# Autodesk Inventor assembly: メカオンリーiam
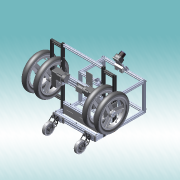
[picture p0: Inventor's stored thumbnail of the model, 180x180]
Saved by Autodesk Inventor 2015 (Build 190159000, 159)
## iProperties
Created: 2016-02-29
Part Number: メカオンリーiam
Document SubType Name: Assembly
Designer: buzztaka
Author: buzztaka
## Documents named in this file (51)
- C:\Users\buzztaka\Documents\tukuba\i-cart-middle_3d-model\計測輪アセンブル\メカオンリーiam.iam
- C:\Users\buzztaka\Documents\tukuba\i-cart-middle_3d-model\計測輪アセンブル\wheel_12inch.ipt
- C:\Users\buzztaka\Documents\tukuba\i-cart-middle_3d-model\計測輪アセンブル\wheel-cap.ipt
- C:\Users\buzztaka\Documents\tukuba\i-cart-middle_3d-model\計測輪アセンブル\wheel-hub.ipt
- C:\Users\buzztaka\Documents\tukuba\i-cart-middle_3d-model\計測輪アセンブル\HFS60A5-20-70.ipt
- C:\Users\buzztaka\Documents\tukuba\i-cart-middle_3d-model\計測輪アセンブル\HBLBL5.ipt
- C:\Users\buzztaka\Documents\tukuba\i-cart-middle_3d-model\計測輪アセンブル\hblfsn5.ipt
- C:\Users\buzztaka\Documents\tukuba\i-cart-middle_3d-model\計測輪アセンブル\hblfsnf5.ipt
- C:\Users\buzztaka\Documents\tukuba\i-cart-middle_3d-model\計測輪アセンブル\HBLFSSW5.ipt
- C:\Users\buzztaka\Documents\tukuba\i-cart-middle_3d-model\計測輪アセンブル\hntaj5_5.ipt
- C:\Users\buzztaka\Documents\tukuba\i-cart-middle_3d-model\計測輪アセンブル\UST-20LX.ipt
- C:\Users\buzztaka\Documents\tukuba\i-cart-middle_3d-model\計測輪アセンブル\MTi-30.ipt
- C:\Users\buzztaka\Documents\tukuba\i-cart-middle_3d-model\計測輪アセンブル\HFSB5-2020-550-LCH-RWV-AH30-BH240-CH280-DH442-EH462.ipt
- C:\Users\buzztaka\Documents\tukuba\i-cart-middle_3d-model\計測輪アセンブル\CAF5-2020-432-LCH-RCH-AH167-BH217.ipt
- C:\Users\buzztaka\Documents\tukuba\i-cart-middle_3d-model\計測輪アセンブル\エンコーダ取り付け.iam
- C:\Users\buzztaka\Documents\tukuba\i-cart-middle_3d-model\計測輪アセンブル\HFSB5-2020-80-TPW.ipt
- C:\Users\buzztaka\Documents\tukuba\i-cart-middle_3d-model\計測輪アセンブル\CAF5-2040-432-LCH-RCH-AH167-BH217切り出し後.ipt
- C:\Users\buzztaka\Documents\tukuba\i-cart-middle_3d-model\計測輪アセンブル\ힼ�ힼ�ힼ�ힼ�.ipt
- C:\Users\buzztaka\Documents\tukuba\i-cart-middle_3d-model\計測輪アセンブル\ힼ�ힼ�ힼ�ힼ�ힼ�-L1.ipt
- C:\Users\buzztaka\Documents\tukuba\i-cart-middle_3d-model\計測輪アセンブル\ힼ�ힼ�ힼ�ힼ�ힼ�-L2.ipt
- C:\Users\buzztaka\Documents\tukuba\i-cart-middle_3d-model\計測輪アセンブル\ힼ�ힼ�ힼ�ힼ�ힼ�-ힽ�ힽ�.ipt
- C:\Users\buzztaka\Documents\tukuba\i-cart-middle_3d-model\計測輪アセンブル\ힼ�ힼ�ힼ�ힼ�ힼ�-ힼ�ힽ�ힽ�.ipt
- C:\Users\buzztaka\Documents\tukuba\i-cart-middle_3d-model\計測輪アセンブル\ힼ�ힼ�ힼ�ힼ�-ힼ�ힽ�ힽ�Lힼ�ힼ�ힼ�ힼ�ힼ�.ipt
- C:\Users\buzztaka\Documents\tukuba\i-cart-middle_3d-model\計測輪アセンブル\ힼ�ힼ�ힼ�ힼ�ힼ�-ힼ�ힼ�ힼ�ힼ�ힼ�ힽ�ힼ�ힼ�ힽ�.ipt
- C:\Users\buzztaka\Documents\tukuba\i-cart-middle_3d-model\計測輪アセンブル\ힼ�ힼ�ힼ�ힼ�(ힽ�ힽ�).ipt
- C:\Users\buzztaka\Documents\tukuba\i-cart-middle_3d-model\計測輪アセンブル\ힼ�ힼ�ힼ�ힼ�ힼ�ힼ�ힼ�-2020-L2.ipt
- C:\Users\buzztaka\Documents\tukuba\i-cart-middle_3d-model\計測輪アセンブル\ힼ�ힼ�ힼ�ힼ�ힼ�ힼ�ힼ�-2040-L2.ipt
- C:\Users\buzztaka\Documents\tukuba\i-cart-middle_3d-model\計測輪アセンブル\ힼ�ힼ�ힼ�ힼ�ힼ�ힼ�ힼ�-2060-L2.ipt
- C:\Users\buzztaka\Documents\tukuba\i-cart-middle_3d-model\計測輪アセンブル\ힼ�ힼ�ힼ�ힼ�ힼ�ힼ�ힼ�-2040-L3.ipt
- C:\Users\buzztaka\Documents\tukuba\i-cart-middle_3d-model\計測輪アセンブル\ힼ�ힼ�ힼ�ힼ�ힼ�ힼ�ힼ�-2020-L4.ipt
- C:\Users\buzztaka\Documents\tukuba\i-cart-middle_3d-model\計測輪アセンブル\ힼ�ힼ�ힼ�ힼ�ힼ�ힼ�ힼ�-2020-L5.ipt
- C:\Users\buzztaka\Documents\tukuba\i-cart-middle_3d-model\計測輪アセンブル\ힼ�ힼ�ힼ�ힼ�ힼ�ힼ�ힼ�-2020-L6.ipt
- C:\Users\buzztaka\Documents\tukuba\i-cart-middle_3d-model\計測輪アセンブル\ힼ�ힼ�ힼ�ힼ�ힼ�ힼ�ힼ�-2020-L7.ipt
- C:\Users\buzztaka\Documents\tukuba\i-cart-middle_3d-model\計測輪アセンブル\ힼ�ힼ�ힼ�ힼ�ힼ�ힼ�ힼ�-ힽ�ힽ�ힽ�ힼ�ힼ�ힼ�ힼ�ힼ�ힼ�.ipt
- C:\Users\buzztaka\Documents\tukuba\i-cart-middle_3d-model\計測輪アセンブル\ힼ�ힼ�ힼ�ힼ�ힼ�ힼ�ힼ�-ힼ�ힼ�ힼ�-M5.ipt
- C:\Users\buzztaka\Documents\tukuba\i-cart-middle_3d-model\計測輪アセンブル\ힼ�ힼ�ힼ�ힼ�ힼ�ힼ�ힼ�-ힽ�ힼ�ힽ�ힼ�ힼ�.ipt
- C:\Users\buzztaka\Documents\tukuba\i-cart-middle_3d-model\計測輪アセンブル\URG_ힼ�ힽ�ힽ�ힼ�ힼ�ힼ�ힽ�.ipt
- C:\Users\buzztaka\Documents\tukuba\i-cart-middle_3d-model\計測輪アセンブル\imu_ힼ�ힼ�ힼ�ힼ�.ipt
- C:\Users\buzztaka\Documents\tukuba\i-cart-middle_3d-model\計測輪アセンブル\ힽ�ힼ�ힼ�ힼ�ힼ�ힽ�.ipt
- C:\Users\buzztaka\Documents\tukuba\i-cart-middle_3d-model\計測輪アセンブル\M3ힽ�ힼ�ힼ�ힼ�ힼ�ힼ�ힼ�.ipt
- C:\Users\buzztaka\Documents\tukuba\i-cart-middle_3d-model\計測輪アセンブル\ힼ�ힼ�ힼ�-M5.ipt
- C:\Users\buzztaka\Documents\tukuba\i-cart-middle_3d-model\計測輪アセンブル\ힼ�ힼ�-Cap-M5-12.ipt
- C:\Users\buzztaka\Documents\tukuba\i-cart-middle_3d-model\計測輪アセンブル\ힼ�ힼ�-Cap-M5-10.ipt
- C:\Users\buzztaka\Documents\tukuba\i-cart-middle_3d-model\計測輪アセンブル\ힼ�ힼ�-Cap-M5-8.ipt
- C:\Users\buzztaka\Documents\tukuba\i-cart-middle_3d-model\計測輪アセンブル\ힼ�ힼ�-ힼ�ힼ�-M5.ipt
- C:\Users\buzztaka\Documents\tukuba\i-cart-middle_3d-model\計測輪アセンブル\ힼ�ힼ�-ힼ�ힼ�-M3.ipt
- C:\Users\buzztaka\Documents\tukuba\i-cart-middle_3d-model\計測輪アセンブル\ힼ�ힼ�-Cap-M3-6.ipt
- C:\Users\buzztaka\Documents\tukuba\i-cart-middle_3d-model\計測輪アセンブル\ힼ�ힼ�-Cap-M5-60.ipt
- C:\Users\buzztaka\Documents\tukuba\i-cart-middle_3d-model\計測輪アセンブル\ힼ�ힼ�-Cap-M6-10.ipt
- C:\Users\buzztaka\Documents\tukuba\i-cart-middle_3d-model\計測輪アセンブル\ힼ�ힼ�-ힼ�ힼ�ힼ�-M3-16.ipt
- C:\Users\buzztaka\Documents\tukuba\i-cart-middle_3d-model\計測輪アセンブル\ힼ�ힼ�ힽ�-M5.ipt
## Components (68 placed, 16 different names)
1. wheel_12inch
2. wheel-cap
3. wheel-hub
4. HFS60A5-20-70
5. HBLBL5
6. hblfsn5
7. hblfsnf5
8. hblfsnf5:1
9. hblfsnf5:2
10. HBLFSSW5
11. hntaj5_5
12. hntaj5_5:1
13. hntaj5_5:2
14. hntaj5_5:3
15. hntaj5_5:4
16. hntaj5_5:5
17. hntaj5_5:6
18. hntaj5_5:7
19. hntaj5_5:8
20. hntaj5_5:9
21. hntaj5_5:10
22. hntaj5_5:11
23. hntaj5_5:12
24. hntaj5_5:16
25. hntaj5_5:17
26. hntaj5_5:18
27. hntaj5_5:19
28. hntaj5_5:20
29. hntaj5_5:21
30. hntaj5_5:22
31. hntaj5_5:23
32. hntaj5_5:24
33. hntaj5_5:25
34. wheel_12inch:1
35. wheel-cap:1
36. wheel-hub:1
37. UST-20LX
38. MTi-30
39. HBLBL5:1
40. hblfsn5:1
41. hblfsnf5:3
42. hblfsnf5:4
43. hntaj5_5:26
44. hntaj5_5:27
45. hntaj5_5:28
46. hntaj5_5:29
47. hntaj5_5:30
48. hntaj5_5:31
49. hntaj5_5:32
50. hntaj5_5:33
51. hntaj5_5:35
52. hntaj5_5:36
53. hntaj5_5:37
54. hntaj5_5:38
55. hntaj5_5:39
56. hntaj5_5:40
57. hntaj5_5:41
58. hntaj5_5:42
59. HFSB5-2020-550-LCH-RWV-AH30-BH240-CH280-DH442-EH462:1 — 挿入:1, 挿入:2, 挿入:5, 挿入:20, 挿入:21
60. HFSB5-2020-550-LCH-RWV-AH30-BH240-CH280-DH442-EH462:2 — 挿入:3, 挿入:4, 挿入:24, 挿入:25
61. CAF5-2020-432-LCH-RCH-AH167-BH217:2 — 挿入:18, 挿入:19, 挿入:22, 挿入:23
62. エンコーダ取り付け:1 [sub-assembly] — 挿入:18, 挿入:19, 挿入:30
63. HFSB5-2020-80-TPW:1 — 挿入:24, 挿入:27
64. HFSB5-2020-80-TPW:2 — 挿入:25, 挿入:26
65. HFSB5-2020-80-TPW:3 — 挿入:20, 挿入:22
66. HFSB5-2020-80-TPW:4 — 挿入:21, 挿入:23
67. CAF5-2040-432-LCH-RCH-AH167-BH217切り出し後:1 — 挿入:26, 挿入:27, 挿入:28, 挿入:29
68. エンコーダ取り付け:2 [sub-assembly] — 挿入:28, 挿入:29, 挿入:32
## Relationships (21: Insert 21)
- 挿入:1 [Insert]: HFSB5-2020-550-LCH-RWV-AH30-BH240-CH280-DH442-EH462:1
- 挿入:2 [Insert]: HFSB5-2020-550-LCH-RWV-AH30-BH240-CH280-DH442-EH462:1
- 挿入:3 [Insert]: HFSB5-2020-550-LCH-RWV-AH30-BH240-CH280-DH442-EH462:2
- 挿入:4 [Insert]: HFSB5-2020-550-LCH-RWV-AH30-BH240-CH280-DH442-EH462:2
- 挿入:5 [Insert]: HFSB5-2020-550-LCH-RWV-AH30-BH240-CH280-DH442-EH462:1
- 挿入:18 [Insert]: CAF5-2020-432-LCH-RCH-AH167-BH217:2 ↔ エンコーダ取り付け:1
- 挿入:19 [Insert]: CAF5-2020-432-LCH-RCH-AH167-BH217:2 ↔ エンコーダ取り付け:1
- 挿入:20 [Insert]: HFSB5-2020-550-LCH-RWV-AH30-BH240-CH280-DH442-EH462:1 ↔ HFSB5-2020-80-TPW:3
- 挿入:21 [Insert]: HFSB5-2020-550-LCH-RWV-AH30-BH240-CH280-DH442-EH462:1 ↔ HFSB5-2020-80-TPW:4
- 挿入:22 [Insert]: CAF5-2020-432-LCH-RCH-AH167-BH217:2 ↔ HFSB5-2020-80-TPW:3
- 挿入:23 [Insert]: CAF5-2020-432-LCH-RCH-AH167-BH217:2 ↔ HFSB5-2020-80-TPW:4
- 挿入:24 [Insert]: HFSB5-2020-550-LCH-RWV-AH30-BH240-CH280-DH442-EH462:2 ↔ HFSB5-2020-80-TPW:1
- 挿入:25 [Insert]: HFSB5-2020-550-LCH-RWV-AH30-BH240-CH280-DH442-EH462:2 ↔ HFSB5-2020-80-TPW:2
- 挿入:26 [Insert]: HFSB5-2020-80-TPW:2 ↔ CAF5-2040-432-LCH-RCH-AH167-BH217切り出し後:1
- 挿入:27 [Insert]: HFSB5-2020-80-TPW:1 ↔ CAF5-2040-432-LCH-RCH-AH167-BH217切り出し後:1
- 挿入:28 [Insert]: CAF5-2040-432-LCH-RCH-AH167-BH217切り出し後:1 ↔ エンコーダ取り付け:2
- 挿入:29 [Insert]: CAF5-2040-432-LCH-RCH-AH167-BH217切り出し後:1 ↔ エンコーダ取り付け:2
- 挿入:30 [Insert]: エンコーダ取り付け:1
- 挿入:31 [Insert]
- 挿入:32 [Insert]: エンコーダ取り付け:2
- 挿入:33 [Insert]
